# Autodesk Inventor assembly: SolarPanel
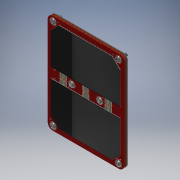
[picture p0: Inventor's stored thumbnail of the model, 180x180]
Saved by Autodesk Inventor 2018 (Build 220112000, 112)
## iProperties
Created: 2018-05-13
Part Number: SolarPanel
Document SubType Name: Assembly
Designer: Bradley
Author: Bradley
## Documents named in this file (9)
- D:\Users\Bradley\Documents\CougsInSpace\CougSat1-Hardware\CougSat1-PowerBoard\CADModel\Native\SolarPanel-X.iam
- D:\Users\Bradley\Documents\CougsInSpace\CougSat1-Hardware\CougSat1-PowerBoard\CADModel\Native\SolarPanel_PCB.ipt
- D:\Users\Bradley\Documents\CougsInSpace\CougSat1-Hardware\CougSat1-PowerBoard\CADModel\Native\SolarPanel_CoilForm.ipt
- D:\Users\Bradley\Documents\CougsInSpace\Resources\ComponentModels\Electronics\SolarCell_UTJ.ipt
- D:\Users\Bradley\Documents\CougsInSpace\Resources\ComponentModels\Fasteners\Bolt_M3x0.35_8mm_BH.ipt
- D:\Users\Bradley\Documents\CougsInSpace\Resources\ComponentModels\Fasteners\Bolt_M3x0.35_10mm_BH.ipt
- D:\Users\Bradley\Documents\CougsInSpace\CougSat1-Hardware\CougSat1-PowerBoard\CADModel\Native\SolarPanel_Coil.ipt
- D:\Users\Bradley\Documents\CougsInSpace\Resources\ComponentModels\Connectors\PicoLock-J-10.ipt
- D:\Users\Bradley\Documents\CougsInSpace\Resources\ComponentModels\Connectors\PicoLock-P-10.ipt
## Components (13 placed, 8 different names)
1. SolarPanel_CoilForm:1 — Insert:1, Insert:2, Insert:9, Insert:10
2. SolarPanel_PCB:1 — Insert:1, Insert:2, Insert:3, Insert:4, Insert:5, Insert:6, Insert:7, Insert:8, Mate:1, Mate:2, Mate:7, Flush:4, Flush:5
3. SolarPanel_Coil:1 — Insert:9, Insert:10
4. PicoLock-J-10:1 — Mate:7, Flush:4, Flush:5
5. PicoLock-P-10:1
6. SolarCell_UTJ:1 — Mate:1, Flush:1, Flush:2
7. SolarCell_UTJ:2 — Mate:2, Mate:3, Mate:4
8. Bolt_M3x0.35_10mm_BH:1 — Insert:5
9. Bolt_M3x0.35_10mm_BH:2 — Insert:6
10. Bolt_M3x0.35_8mm_BH:1 — Insert:7
11. Bolt_M3x0.35_8mm_BH:2 — Insert:8
12. Bolt_M3x0.35_8mm_BH:3 — Insert:3
13. Bolt_M3x0.35_8mm_BH:4 — Insert:4
## Relationships (22: Insert 10, Mate 7, Flush 5)
- Insert:1: SolarPanel_CoilForm:1 ↔ SolarPanel_PCB:1
- Insert:2: SolarPanel_CoilForm:1 ↔ SolarPanel_PCB:1
- Insert:3: SolarPanel_PCB:1 ↔ Bolt_M3x0.35_8mm_BH:3
- Insert:4: SolarPanel_PCB:1 ↔ Bolt_M3x0.35_8mm_BH:4
- Insert:5: SolarPanel_PCB:1 ↔ Bolt_M3x0.35_10mm_BH:1
- Insert:6: SolarPanel_PCB:1 ↔ Bolt_M3x0.35_10mm_BH:2
- Insert:7: SolarPanel_PCB:1 ↔ Bolt_M3x0.35_8mm_BH:1
- Insert:8: SolarPanel_PCB:1 ↔ Bolt_M3x0.35_8mm_BH:2
- Mate:1: SolarPanel_PCB:1 ↔ SolarCell_UTJ:1
- Mate:2: SolarPanel_PCB:1 ↔ SolarCell_UTJ:2
- Flush:1: SolarCell_UTJ:1
- Mate:3: SolarCell_UTJ:2
- Mate:4 (5 mm): SolarCell_UTJ:2
- Flush:2 (5 mm): SolarCell_UTJ:1
- Insert:9: SolarPanel_CoilForm:1 ↔ SolarPanel_Coil:1
- Insert:10: SolarPanel_CoilForm:1 ↔ SolarPanel_Coil:1
- [Mate] (0.025 mm): PicoLock-J-10:1 ↔ PicoLock-P-10:1
- [Mate]: PicoLock-J-10:1 ↔ PicoLock-P-10:1
- [Flush]: PicoLock-J-10:1 ↔ PicoLock-P-10:1
- Mate:7: SolarPanel_PCB:1 ↔ PicoLock-J-10:1
- Flush:4 (0.15 mm): SolarPanel_PCB:1 ↔ PicoLock-J-10:1
- Flush:5 (0.15 mm): SolarPanel_PCB:1 ↔ PicoLock-J-10:1
